# Autodesk Inventor assembly: Assembly1
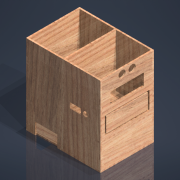
[picture p0: Inventor's stored thumbnail of the model, 180x180]
Saved by Autodesk Inventor 2021 (Build 250183000, 183)
## iProperties
Created: 2020-11-18
Part Number: Assembly1
Document SubType Name: Assembly
Designer: riley
Author: riley
## Documents named in this file (7)
- C:\Users\riley\Documents\0 COVID Bot\Assembly1.iam
- C:\Users\riley\Documents\0 COVID Bot\Base Plate.ipt
- C:\Users\riley\Documents\0 COVID Bot\Sideplate.ipt
- C:\Users\riley\Documents\0 COVID Bot\Fascia.ipt
- C:\Users\riley\Documents\0 COVID Bot\Fascia2.ipt
- C:\Users\riley\Documents\0 COVID Bot\Sideplate2.ipt
- C:\Users\riley\Documents\0 COVID Bot\Door.ipt
## Components (8 placed, 6 different names)
1. Base Plate:1 — Flush:1, Mate:5, Flush:5, Flush:6, Flush:14, Flush:15, Flush:16, Flush:17, Flush:18
2. Sideplate:1 — Flush:1, Flush:9, Mate:9, Flush:13
3. Base Plate:2 — Mate:5, Flush:5, Flush:6, Mate:6, Mate:7, Flush:10, Mate:8
4. Fascia:2 — Mate:6, Mate:7, Flush:9
5. Fascia:3 — Flush:10, Flush:14, Flush:15
6. Fascia2:1 — Mate:8, Mate:9, Flush:13, Flush:19
7. Sideplate2:1 — Flush:16, Flush:17, Flush:18
8. Door:1 — Flush:19
## Relationships (17: Flush 12, Mate 5)
- Flush:1: Base Plate:1 ↔ Sideplate:1
- Mate:5 (50.8 mm): Base Plate:1 ↔ Base Plate:2
- Flush:5: Base Plate:1 ↔ Base Plate:2
- Flush:6: Base Plate:1 ↔ Base Plate:2
- Mate:6: Base Plate:2 ↔ Fascia:2
- Mate:7: Base Plate:2 ↔ Fascia:2
- Flush:9: Sideplate:1 ↔ Fascia:2
- Flush:10: Base Plate:2 ↔ Fascia:3
- Mate:8: Base Plate:2 ↔ Fascia2:1
- Mate:9: Sideplate:1 ↔ Fascia2:1
- Flush:13: Sideplate:1 ↔ Fascia2:1
- Flush:14: Base Plate:1 ↔ Fascia:3
- Flush:15: Base Plate:1 ↔ Fascia:3
- Flush:16: Base Plate:1 ↔ Sideplate2:1
- Flush:17: Base Plate:1 ↔ Sideplate2:1
- Flush:18: Base Plate:1 ↔ Sideplate2:1
- Flush:19: Fascia2:1 ↔ Door:1
